# Autodesk Inventor assembly: assembly
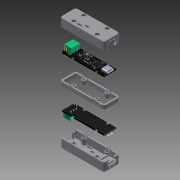
[picture p0: Inventor's stored thumbnail of the model, 180x180]
Saved by Autodesk Inventor 2014 SP2 (Build 180246200, 246)
## iProperties
Created: 2025-01-20
Part Number: assembly
Document SubType Name: Assembly
Designer: GauchoHP
Author: GauchoHP
## Documents named in this file (4)
- E:\Dati\Documenti_Emanuele\Linguaggi_di_Programmazione\ST MCU\baccable\canable\CANableAndLedsStripController\hardware\box\fysect ucan\assembly.iam
- E:\Dati\Documenti_Emanuele\Linguaggi_di_Programmazione\ST MCU\baccable\canable\CANableAndLedsStripController\hardware\box\fysect ucan\dualBaccable-ucan_fysect.ipt
- E:\Dati\Documenti_Emanuele\Linguaggi_di_Programmazione\ST MCU\baccable\canable\CANableAndLedsStripController\hardware\box\fysect ucan\Imported Components\UCAN_ V1.0\UCAN_ V1.0.iam
- E:\Dati\Documenti_Emanuele\Linguaggi_di_Programmazione\ST MCU\baccable\canable\CANableAndLedsStripController\hardware\box\fysect ucan\dualBaccable-ucan_fysect_middle.ipt
## Components (5 placed, 3 different names)
1. dualBaccable-ucan_fysect:1 — Mate:1, Mate:2, Mate:3
2. dualBaccable-ucan_fysect:2 — Mate:10, Mate:11, Mate:12
3. UCAN_ V1.0:1 [sub-assembly] — Mate:1, Mate:2, Mate:3, Mate:4, Mate:5, Mate:6
4. UCAN_ V1.0:2 [sub-assembly] — Mate:7, Mate:8, Mate:9, Mate:10, Mate:11, Mate:12
5. dualBaccable-ucan_fysect_middle:1 — Mate:4, Mate:5, Mate:6, Mate:7, Mate:8, Mate:9
## Relationships (12: Mate 12)
- Mate:1: dualBaccable-ucan_fysect:1 ↔ UCAN_ V1.0:1
- Mate:2 (0.1 mm): dualBaccable-ucan_fysect:1 ↔ UCAN_ V1.0:1
- Mate:3 (30 mm): dualBaccable-ucan_fysect:1 ↔ UCAN_ V1.0:1
- Mate:4: UCAN_ V1.0:1 ↔ dualBaccable-ucan_fysect_middle:1
- Mate:5 (0.1 mm): UCAN_ V1.0:1 ↔ dualBaccable-ucan_fysect_middle:1
- Mate:6 (30 mm): UCAN_ V1.0:1 ↔ dualBaccable-ucan_fysect_middle:1
- Mate:7: UCAN_ V1.0:2 ↔ dualBaccable-ucan_fysect_middle:1
- Mate:8 (0.1 mm): UCAN_ V1.0:2 ↔ dualBaccable-ucan_fysect_middle:1
- Mate:9 (30 mm): UCAN_ V1.0:2 ↔ dualBaccable-ucan_fysect_middle:1
- Mate:10: dualBaccable-ucan_fysect:2 ↔ UCAN_ V1.0:2
- Mate:11 (0.1 mm): dualBaccable-ucan_fysect:2 ↔ UCAN_ V1.0:2
- Mate:12 (30 mm): dualBaccable-ucan_fysect:2 ↔ UCAN_ V1.0:2
